# Autodesk Inventor assembly: ToASI-0B
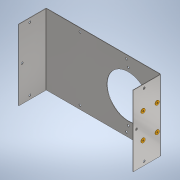
[picture p0: Inventor's stored thumbnail of the model, 180x180]
Saved by Autodesk Inventor 2020.3 (Build 243373000, 373)
## iProperties
Created: 2020-07-31
Part Number: ToASI-0B
Document SubType Name: Assembly
Designer: Bruno
Author: Bruno
## Documents named in this file (3)
- C:\Users\Bruno\Desktop\Github\CAD\Inventor\For ASI\ToASI-0B.iam
- C:\Users\Bruno\Desktop\Github\CAD\Inventor\Heater-Box\Box-Disk\Box top.ipt
- C:\Users\Bruno\Desktop\Github\CAD\Inventor\Heater-Box\Box-Disk\M4 Rivet nut.ipt
## Components (5 placed, 2 different names)
1. Box top:1 — Cylindrical:1, Cylindrical:2, Cylindrical:3, Cylindrical:4
2. M4 Rivet nut:1 — Cylindrical:1
3. M4 Rivet nut:2 — Cylindrical:3
4. M4 Rivet nut:3 — Cylindrical:4
5. M4 Rivet nut:4 — Cylindrical:2
## Relationships (4: CylindricalJoint 4)
- Cylindrical:1: Box top:1 ↔ M4 Rivet nut:1
- Cylindrical:2: Box top:1 ↔ M4 Rivet nut:4
- Cylindrical:3: Box top:1 ↔ M4 Rivet nut:2
- Cylindrical:4: Box top:1 ↔ M4 Rivet nut:3
